# Autodesk Inventor assembly: Сборка_Датчик
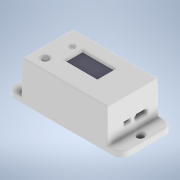
[picture p0: Inventor's stored thumbnail of the model, 180x180]
Saved by Autodesk Inventor 2022 (Build 260153000, 153)
## iProperties
Created: 2022-01-08
Part Number: Сборка_Датчик
Document SubType Name: Assembly
Designer: Me
Author: Me
## Documents named in this file (5)
- C:\Users\Me\Documents\Сборка_Датчик.iam
- C:\Users\Me\Documents\case_down.ipt
- C:\Users\Me\Documents\803040-950.ipt
- C:\Users\Me\Documents\case_up.ipt
- C:\Users\Me\Documents\step_pcb\Curse_PCB.iam
## Components (4 placed, 4 different names)
1. case_down:1 — Совмещение:1, Совмещение:2, Совмещение:3, Совмещение:4, Совмещение:5, Совмещение:6, Плоский:1
2. 803040-950:1 — Совмещение:1, Совмещение:2, Совмещение:3
3. case_up:1 — Совмещение:4, Совмещение:5, Совмещение:6
4. Curse_PCB:1 [sub-assembly] — Плоский:1
## Relationships (7: Mate 6, PlanarJoint 1)
- Совмещение:1 [Mate] (6 mm): case_down:1 ↔ 803040-950:1
- Совмещение:2 [Mate] (0.5 mm): case_down:1 ↔ 803040-950:1
- Совмещение:3 [Mate] (0.1 mm): case_down:1 ↔ 803040-950:1
- Совмещение:4 [Mate]: case_down:1 ↔ case_up:1
- Совмещение:5 [Mate] (1 mm): case_down:1 ↔ case_up:1
- Совмещение:6 [Mate] (1 mm): case_down:1 ↔ case_up:1
- Плоский:1 [PlanarJoint] (11.6 mm): case_down:1 ↔ Curse_PCB:1
